# Autodesk Inventor assembly: temp
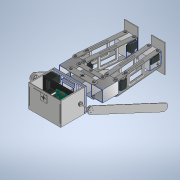
[picture p0: Inventor's stored thumbnail of the model, 180x180]
Saved by Autodesk Inventor 2022 (Build 260153000, 153)
## iProperties
Created: 2022-10-09
Part Number: temp
Document SubType Name: Assembly
Designer: haya
Author: haya
## Documents named in this file (48)
- C:\Users\haya\Documents\GitHub\reduce_joint\reduce_joint.iam
- C:\Users\haya\Documents\GitHub\reduce_joint\foot_link.ipt
- C:\Users\haya\Documents\GitHub\reduce_joint\B3M10xx.ipt
- B3M11xx.ipt
- C:\Users\haya\Documents\GitHub\reduce_joint\ankle.ipt
- C:\Users\haya\Documents\GitHub\reduce_joint\CC-2230-25B.ipt
- C:\Users\haya\Documents\GitHub\reduce_joint\CC-2230-10B.ipt
- C:\Users\haya\Documents\GitHub\reduce_joint\foot.ipt
- C:\Users\haya\Documents\GitHub\reduce_joint\hip.ipt
- C:\Users\haya\Documents\GitHub\reduce_joint\hip_servo_jig.ipt
- C:\Users\haya\Documents\GitHub\reduce_joint\hip_link.ipt
- C:\Users\haya\Documents\GitHub\reduce_joint\crotch.ipt
- C:\Users\haya\Documents\GitHub\reduce_joint\joint.iam
- C:\Users\haya\Documents\GitHub\reduce_joint\waist1..ipt
- C:\Users\haya\Documents\GitHub\reduce_joint\waist2.ipt
- C:\Users\haya\Documents\GitHub\reduce_joint\GEFHBS0_5-50-3-10-W0_b.ipt
- C:\Users\haya\Documents\GitHub\reduce_joint\GEABS0_5-80-2-B-5_b.ipt
- C:\Users\haya\Documents\GitHub\reduce_joint\80F-0505.ipt
- C:\Users\haya\Documents\GitHub\reduce_joint\arm_shaft.ipt
- C:\Users\haya\Documents\GitHub\reduce_joint\body_left.ipt
- C:\Users\haya\Documents\GitHub\reduce_joint\body_right.ipt
- C:\Users\haya\Documents\GitHub\reduce_joint\SSCSJ5-6b.ipt
- C:\Users\haya\Documents\GitHub\reduce_joint\既製品\バッテリー(G7 HI-VOLTAGE 2400MAH 3S 75CMAX LIPO).ipt
- C:\Users\haya\Documents\GitHub\reduce_joint\body_top.ipt
- C:\Users\haya\Documents\GitHub\reduce_joint\raspberrypi_b_+_(assembly)\raspberrypi_b_+_(assembly).iam
- C:\Users\haya\Documents\GitHub\reduce_joint\circuit_base.ipt
- C:\Users\haya\Documents\GitHub\reduce_joint\SCMW5b.ipt
- C:\Users\haya\Documents\GitHub\reduce_joint\arm_link.ipt
- C:\Users\haya\Documents\GitHub\reduce_joint\head.ipt
- C:\Users\haya\Documents\GitHub\reduce_joint\center_servo_jig.ipt
- C:\Users\haya\Documents\GitHub\reduce_joint\lever.ipt
- C:\Users\haya\Documents\GitHub\reduce_joint\foot_link_lever.ipt
- C:\Users\haya\Documents\GitHub\reduce_joint\joint_hip.iam
- C:\Users\haya\Documents\GitHub\reduce_joint\hip_link_motor.ipt
- C:\Users\haya\Documents\GitHub\reduce_joint\foot_connect.ipt
- C:\Users\haya\Documents\GitHub\reduce_joint\foot_link_lever_MIR.ipt
- C:\Users\haya\Documents\GitHub\reduce_joint\B3M10xx_MIR.ipt
- C:\Users\haya\Documents\GitHub\reduce_joint\ankle_MIR.ipt
- C:\Users\haya\Documents\GitHub\reduce_joint\CC-2230-25B_MIR.ipt
- C:\Users\haya\Documents\GitHub\reduce_joint\CC-2230-10B_MIR.ipt
- C:\Users\haya\Documents\GitHub\reduce_joint\foot_MIR.ipt
- C:\Users\haya\Documents\GitHub\reduce_joint\hip_MIR2.ipt
- C:\Users\haya\Documents\GitHub\reduce_joint\foot_link_MIR.ipt
- C:\Users\haya\Documents\GitHub\reduce_joint\hip_servo_jig_MIR.ipt
- C:\Users\haya\Documents\GitHub\reduce_joint\joint_MIR.iam
- C:\Users\haya\Documents\GitHub\reduce_joint\lever_MIR.ipt
- C:\Users\haya\Documents\GitHub\reduce_joint\joint_hip_MIR.iam
- C:\Users\haya\Documents\GitHub\reduce_joint\foot_connect_MIR.ipt
## Components (87 placed, 46 different names)
1. foot_link_lever:1 — 角度:6, 挿入:110, 挿入:111, 正接:1, フラッシュ:16, メイト:26, 角度:11
2. B3M11xx:1 — 角度:1, 挿入:4, 挿入:7
3. ankle:1 — 角度:1, 挿入:4, 挿入:5, 挿入:81, 挿入:82, 角度:2, 挿入:113, 挿入:114
4. CC-2230-25B:1 — 挿入:5, 挿入:6
5. CC-2230-10B:1 — 挿入:6
6. foot:1 — 挿入:7, 角度:2
7. hip:1 — メイト:1, フラッシュ:1, メイト:2, 挿入:77, 挿入:78, 挿入:85, 挿入:86, 角度:6, 挿入:116, 挿入:118, 挿入:121, 挿入:122, 角度:11
8. foot_link:2 — 挿入:84, 挿入:88, メイト:28
9. B3M11xx:2 — フラッシュ:2, メイト:3, フラッシュ:3, 挿入:109
10. hip_servo_jig:1 — メイト:1, フラッシュ:1, メイト:2, フラッシュ:2, メイト:3, フラッシュ:3
11. hip_link:1 — 挿入:72, 挿入:76, 挿入:80, 角度:10
12. hip_link_motor:1 — 挿入:71, 挿入:79, メイト:8
13. crotch:1 — 挿入:74, フラッシュ:4, メイト:4, メイト:5, メイト:7, メイト:8, 角度:3, メイト:9, フラッシュ:5, メイト:10, メイト:11, フラッシュ:6, メイト:12, 挿入:123, 挿入:124, 角度:10
14. joint:1 [sub-assembly] — 挿入:71, 挿入:153
15. joint:2 [sub-assembly] — 挿入:72, 挿入:154
16. joint:3 [sub-assembly] — 挿入:74, 挿入:76
17. joint:4 [sub-assembly] — 挿入:77, 挿入:79
18. joint:6 [sub-assembly] — 挿入:78, 挿入:80
19. joint:7 [sub-assembly] — 挿入:82, 挿入:84
20. joint:8 [sub-assembly] — 挿入:81, 挿入:110
21. joint:9 [sub-assembly] — 挿入:86, 挿入:88
22. joint:10 [sub-assembly] — 挿入:85, 挿入:111
23. B3M11xx:3 — メイト:6, メイト:7, 角度:3
24. center_servo_jig:1 — フラッシュ:4, メイト:4, メイト:5, メイト:6
25. waist1.:1 — メイト:11, フラッシュ:6, メイト:12, メイト:17, フラッシュ:11
26. waist2:1 — メイト:9, フラッシュ:5, メイト:10, メイト:13, フラッシュ:7, フラッシュ:8, メイト:15, メイト:16, フラッシュ:9, フラッシュ:10, フラッシュ:14, メイト:21, 角度:13
27. body_left:1 — メイト:13, フラッシュ:7, フラッシュ:8, 挿入:92, 挿入:93, 挿入:94, 挿入:96, メイト:19, フラッシュ:12, フラッシュ:13, メイト:20
28. B3M11xx:4 — メイト:15, 挿入:94, 挿入:95
29. GEFHBS0_5-50-3-10-W0_b:1 — 挿入:95
30. GEABS0_5-80-2-B-5_b:1 — 挿入:92
31. 80F-0505:1 — 挿入:93
32. arm_shaft:1 — 挿入:96, 挿入:100, 挿入:105
33. body_right:1 — メイト:16, フラッシュ:9, フラッシュ:10, 挿入:97, メイト:18, メイト:23
34. 80F-0505:2 — 挿入:97, 挿入:98
35. SSCSJ5-6b:1 — 挿入:98
36. バッテリー(G7 HI-VOLTAGE 2400MAH 3S 75CMAX LIPO):1 — メイト:17, フラッシュ:11, メイト:18
37. body_top:1 — メイト:19, フラッシュ:12, フラッシュ:13, 挿入:99, 角度:4
38. raspberrypi_b_+_(assembly):1 [sub-assembly] — メイト:22, フラッシュ:15, メイト:23
39. circuit_base:1 — フラッシュ:14, メイト:20, メイト:21, メイト:22, フラッシュ:15
40. B3M11xx:5 — 挿入:99, 角度:4, 挿入:103, 挿入:104
41. SCMW5b:1 — 挿入:100, メイト:24, 挿入:101, 挿入:102
42. arm_link:1 — メイト:24, 挿入:101, 挿入:102, 角度:5
43. head:1 — 挿入:103, 挿入:104
44. SCMW5b:2 — 挿入:105, 挿入:106, 挿入:107
45. arm_link:2 — 挿入:106, 挿入:107, 角度:5, 角度:13
46. lever:1 — 挿入:109, 挿入:112
47. joint_hip:1 [sub-assembly] — 挿入:112, 正接:1
48. joint:11 [sub-assembly] — 挿入:113, 挿入:115
49. joint:12 [sub-assembly] — 挿入:114, 挿入:119
50. foot_link:3 — 挿入:115, 挿入:117, メイト:25
51. joint:13 [sub-assembly] — 挿入:116, 挿入:117
52. foot_connect:1 — メイト:25, フラッシュ:16, メイト:26
53. foot_link:4 — 挿入:119, 挿入:120, フラッシュ:17, メイト:27
54. joint:14 [sub-assembly] — 挿入:118, 挿入:120
55. foot_connect:2 — フラッシュ:17, メイト:27, メイト:28
56. joint:15 [sub-assembly] — 挿入:122, 挿入:129
57. joint:16 [sub-assembly] — 挿入:124, 挿入:130
58. joint:17 [sub-assembly] — 挿入:121, 挿入:127
59. joint:18 [sub-assembly] — 挿入:123, 挿入:128
60. joint:19 [sub-assembly] — 挿入:155
61. joint:20 [sub-assembly] — 挿入:156
62. hip_link:2 — 挿入:127, 挿入:128
63. hip_link:3 — 挿入:129, 挿入:130
64. foot_link_lever_MIR:1 — 角度:9, 挿入:137, 挿入:141, 正接:2, メイト:32, フラッシュ:21, 角度:12
65. B3M10xx_MIR:1 — 挿入:131, 角度:7, 挿入:134
66. ankle_MIR:1 — 挿入:131, 角度:7, 挿入:132, 角度:8, 挿入:136, 挿入:138, 挿入:145, 挿入:146
67. CC-2230-25B_MIR:1 — 挿入:132, 挿入:133
68. CC-2230-10B_MIR:1 — 挿入:133
69. foot_MIR:1 — 角度:8, 挿入:134
70. hip_MIR2:1 — 角度:9, メイト:30, フラッシュ:20, メイト:31, 挿入:140, 挿入:142, 挿入:149, 挿入:152, 挿入:153, 挿入:154, 挿入:155, 挿入:156, 角度:12
71. foot_link_MIR:1 — 挿入:135, 挿入:139, メイト:34
72. B3M10xx_MIR:2 — フラッシュ:18, メイト:29, フラッシュ:19, 挿入:143
73. hip_servo_jig_MIR:1 — フラッシュ:18, メイト:29, フラッシュ:19, メイト:30, フラッシュ:20, メイト:31
74. joint_MIR:1 [sub-assembly] — 挿入:135, 挿入:136
75. joint_MIR:2 [sub-assembly] — 挿入:137, 挿入:138
76. joint_MIR:3 [sub-assembly] — 挿入:139, 挿入:140
77. joint_MIR:4 [sub-assembly] — 挿入:141, 挿入:142
78. lever_MIR:1 — 挿入:143, 挿入:144
79. joint_hip_MIR:1 [sub-assembly] — 正接:2, 挿入:144
80. joint_MIR:5 [sub-assembly] — 挿入:145, 挿入:147
81. joint_MIR:6 [sub-assembly] — 挿入:146, 挿入:150
82. foot_link_MIR:2 — 挿入:147, 挿入:148, メイト:33
83. joint_MIR:7 [sub-assembly] — 挿入:148, 挿入:149
84. foot_connect_MIR:1 — メイト:32, フラッシュ:21, メイト:33
85. foot_link_MIR:3 — 挿入:150, 挿入:151, メイト:35, フラッシュ:22
86. joint_MIR:8 [sub-assembly] — 挿入:151, 挿入:152
87. foot_connect_MIR:2 — メイト:34, メイト:35, フラッシュ:22
## Relationships (151: Insert 80, Mate 34, Flush 22, Angle 13, Tangent 2)
- 角度:1 [Angle] (0 deg): B3M11xx:1 ↔ ankle:1
- 挿入:4 [Insert]: B3M11xx:1 ↔ ankle:1
- 挿入:5 [Insert]: ankle:1 ↔ CC-2230-25B:1
- 挿入:6 [Insert]: CC-2230-25B:1 ↔ CC-2230-10B:1
- 挿入:7 [Insert]: B3M11xx:1 ↔ foot:1
- メイト:1 [Mate]: hip:1 ↔ hip_servo_jig:1
- フラッシュ:1 [Flush] (20 mm): hip:1 ↔ hip_servo_jig:1
- メイト:2 [Mate] (0.5 mm): hip:1 ↔ hip_servo_jig:1
- フラッシュ:2 [Flush]: B3M11xx:2 ↔ hip_servo_jig:1
- メイト:3 [Mate]: B3M11xx:2 ↔ hip_servo_jig:1
- フラッシュ:3 [Flush] (-8.5 mm): B3M11xx:2 ↔ hip_servo_jig:1
- 挿入:71 [Insert]: hip_link_motor:1 ↔ joint:1
- 挿入:72 [Insert]: hip_link:1 ↔ joint:2
- 挿入:74 [Insert]: crotch:1 ↔ joint:3
- 挿入:76 [Insert]: hip_link:1 ↔ joint:3
- 挿入:77 [Insert]: hip:1 ↔ joint:4
- 挿入:78 [Insert]: hip:1 ↔ joint:6
- 挿入:79 [Insert]: hip_link_motor:1 ↔ joint:4
- 挿入:80 [Insert]: hip_link:1 ↔ joint:6
- 挿入:81 [Insert]: ankle:1 ↔ joint:8
- 挿入:82 [Insert]: ankle:1 ↔ joint:7
- 挿入:84 [Insert]: foot_link:2 ↔ joint:7
- 挿入:85 [Insert]: hip:1 ↔ joint:10
- 挿入:86 [Insert]: hip:1 ↔ joint:9
- 挿入:88 [Insert]: foot_link:2 ↔ joint:9
- 角度:2 [Angle] (0 deg): ankle:1 ↔ foot:1
- フラッシュ:4 [Flush]: crotch:1 ↔ center_servo_jig:1
- メイト:4 [Mate]: crotch:1 ↔ center_servo_jig:1
- メイト:5 [Mate] (0.5 mm): crotch:1 ↔ center_servo_jig:1
- メイト:6 [Mate]: B3M11xx:3 ↔ center_servo_jig:1
- メイト:7 [Mate]: crotch:1 ↔ B3M11xx:3
- メイト:8 [Mate]: hip_link_motor:1 ↔ crotch:1
- 角度:3 [Angle] (0 deg): crotch:1 ↔ B3M11xx:3
- メイト:9 [Mate]: crotch:1 ↔ waist2:1
- フラッシュ:5 [Flush]: crotch:1 ↔ waist2:1
- メイト:10 [Mate]: crotch:1 ↔ waist2:1
- メイト:11 [Mate]: crotch:1 ↔ waist1.:1
- フラッシュ:6 [Flush]: crotch:1 ↔ waist1.:1
- メイト:12 [Mate]: crotch:1 ↔ waist1.:1
- メイト:13 [Mate]: waist2:1 ↔ body_left:1
- フラッシュ:7 [Flush]: waist2:1 ↔ body_left:1
- フラッシュ:8 [Flush]: waist2:1 ↔ body_left:1
- メイト:15 [Mate]: waist2:1 ↔ B3M11xx:4
- 挿入:92 [Insert] (1 mm): body_left:1 ↔ GEABS0_5-80-2-B-5_b:1
- 挿入:93 [Insert]: body_left:1 ↔ 80F-0505:1
- 挿入:94 [Insert]: body_left:1 ↔ B3M11xx:4
- 挿入:95 [Insert]: B3M11xx:4 ↔ GEFHBS0_5-50-3-10-W0_b:1
- 挿入:96 [Insert] (-50 mm): body_left:1 ↔ arm_shaft:1
- メイト:16 [Mate]: waist2:1 ↔ body_right:1
- フラッシュ:9 [Flush]: waist2:1 ↔ body_right:1
- フラッシュ:10 [Flush]: waist2:1 ↔ body_right:1
- 挿入:97 [Insert]: body_right:1 ↔ 80F-0505:2
- 挿入:98 [Insert]: 80F-0505:2 ↔ SSCSJ5-6b:1
- メイト:17 [Mate]: waist1.:1 ↔ バッテリー(G7 HI-VOLTAGE 2400MAH 3S 75CMAX LIPO):1
- フラッシュ:11 [Flush] (5 mm): waist1.:1 ↔ バッテリー(G7 HI-VOLTAGE 2400MAH 3S 75CMAX LIPO):1
- メイト:18 [Mate] (10 mm): body_right:1 ↔ バッテリー(G7 HI-VOLTAGE 2400MAH 3S 75CMAX LIPO):1
- メイト:19 [Mate]: body_left:1 ↔ body_top:1
- フラッシュ:12 [Flush]: body_left:1 ↔ body_top:1
- フラッシュ:13 [Flush]: body_left:1 ↔ body_top:1
- フラッシュ:14 [Flush]: waist2:1 ↔ circuit_base:1
- メイト:20 [Mate]: body_left:1 ↔ circuit_base:1
- メイト:21 [Mate] (40 mm): waist2:1 ↔ circuit_base:1
- メイト:22 [Mate] (5 mm): raspberrypi_b_+_(assembly):1 ↔ circuit_base:1
- フラッシュ:15 [Flush]: raspberrypi_b_+_(assembly):1 ↔ circuit_base:1
- 挿入:99 [Insert]: body_top:1 ↔ B3M11xx:5
- 角度:4 [Angle] (0 deg): body_top:1 ↔ B3M11xx:5
- メイト:23 [Mate] (10 mm): body_right:1 ↔ raspberrypi_b_+_(assembly):1
- 挿入:100 [Insert]: arm_shaft:1 ↔ SCMW5b:1
- メイト:24 [Mate]: SCMW5b:1 ↔ arm_link:1
- 挿入:101 [Insert]: SCMW5b:1 ↔ arm_link:1
- 挿入:102 [Insert]: SCMW5b:1 ↔ arm_link:1
- 挿入:103 [Insert]: B3M11xx:5 ↔ head:1
- 挿入:104 [Insert]: B3M11xx:5 ↔ head:1
- 挿入:105 [Insert]: arm_shaft:1 ↔ SCMW5b:2
- 挿入:106 [Insert]: SCMW5b:2 ↔ arm_link:2
- 挿入:107 [Insert]: SCMW5b:2 ↔ arm_link:2
- 角度:5 [Angle] (0 deg): arm_link:1 ↔ arm_link:2
- 角度:6 [Angle] (0 deg): foot_link_lever:1 ↔ hip:1
- 挿入:109 [Insert]: B3M11xx:2 ↔ lever:1
- 挿入:110 [Insert]: foot_link_lever:1 ↔ joint:8
- 挿入:111 [Insert]: foot_link_lever:1 ↔ joint:10
- 挿入:112 [Insert]: lever:1 ↔ joint_hip:1
- 正接:1 [Tangent]: foot_link_lever:1 ↔ joint_hip:1
- 挿入:113 [Insert]: ankle:1 ↔ joint:11
- 挿入:114 [Insert]: ankle:1 ↔ joint:12
- 挿入:115 [Insert]: joint:11 ↔ foot_link:3
- 挿入:116 [Insert]: hip:1 ↔ joint:13
- 挿入:117 [Insert]: foot_link:3 ↔ joint:13
- メイト:25 [Mate]: foot_link:3 ↔ foot_connect:1
- フラッシュ:16 [Flush] (-6.5 mm): foot_link_lever:1 ↔ foot_connect:1
- メイト:26 [Mate] (64 mm): foot_link_lever:1 ↔ foot_connect:1
- 挿入:118 [Insert]: hip:1 ↔ joint:14
- 挿入:119 [Insert]: joint:12 ↔ foot_link:4
- 挿入:120 [Insert]: foot_link:4 ↔ joint:14
- フラッシュ:17 [Flush] (-6.5 mm): foot_link:4 ↔ foot_connect:2
- メイト:27 [Mate]: foot_link:4 ↔ foot_connect:2
- メイト:28 [Mate] (64 mm): foot_link:2 ↔ foot_connect:2
- 挿入:121 [Insert]: hip:1 ↔ joint:17
- 挿入:122 [Insert]: hip:1 ↔ joint:15
- 挿入:123 [Insert]: crotch:1 ↔ joint:18
- 挿入:124 [Insert]: crotch:1 ↔ joint:16
- 挿入:127 [Insert]: joint:17 ↔ hip_link:2
- 挿入:128 [Insert]: joint:18 ↔ hip_link:2
- 挿入:129 [Insert]: joint:15 ↔ hip_link:3
- 挿入:130 [Insert]: joint:16 ↔ hip_link:3
- 挿入:131 [Insert]: B3M10xx_MIR:1 ↔ ankle_MIR:1
- 角度:7 [Angle] (0 deg): B3M10xx_MIR:1 ↔ ankle_MIR:1
- 挿入:132 [Insert]: ankle_MIR:1 ↔ CC-2230-25B_MIR:1
- 挿入:133 [Insert]: CC-2230-25B_MIR:1 ↔ CC-2230-10B_MIR:1
- 角度:8 [Angle] (0 deg): ankle_MIR:1 ↔ foot_MIR:1
- 挿入:134 [Insert]: B3M10xx_MIR:1 ↔ foot_MIR:1
- 角度:9 [Angle] (0 deg): foot_link_lever_MIR:1 ↔ hip_MIR2:1
- フラッシュ:18 [Flush] (-8.5 mm): B3M10xx_MIR:2 ↔ hip_servo_jig_MIR:1
- メイト:29 [Mate]: B3M10xx_MIR:2 ↔ hip_servo_jig_MIR:1
- フラッシュ:19 [Flush]: B3M10xx_MIR:2 ↔ hip_servo_jig_MIR:1
- メイト:30 [Mate] (0.5 mm): hip_MIR2:1 ↔ hip_servo_jig_MIR:1
- フラッシュ:20 [Flush] (20 mm): hip_MIR2:1 ↔ hip_servo_jig_MIR:1
- メイト:31 [Mate]: hip_MIR2:1 ↔ hip_servo_jig_MIR:1
- 挿入:135 [Insert]: foot_link_MIR:1 ↔ joint_MIR:1
- 挿入:136 [Insert]: ankle_MIR:1 ↔ joint_MIR:1
- 挿入:137 [Insert]: foot_link_lever_MIR:1 ↔ joint_MIR:2
- 挿入:138 [Insert]: ankle_MIR:1 ↔ joint_MIR:2
- 挿入:139 [Insert]: foot_link_MIR:1 ↔ joint_MIR:3
- 挿入:140 [Insert]: hip_MIR2:1 ↔ joint_MIR:3
- 挿入:141 [Insert]: foot_link_lever_MIR:1 ↔ joint_MIR:4
- 挿入:142 [Insert]: hip_MIR2:1 ↔ joint_MIR:4
- 挿入:143 [Insert]: B3M10xx_MIR:2 ↔ lever_MIR:1
- 正接:2 [Tangent]: foot_link_lever_MIR:1 ↔ joint_hip_MIR:1
- 挿入:144 [Insert]: lever_MIR:1 ↔ joint_hip_MIR:1
- 挿入:145 [Insert]: ankle_MIR:1 ↔ joint_MIR:5
- 挿入:146 [Insert]: ankle_MIR:1 ↔ joint_MIR:6
- 挿入:147 [Insert]: joint_MIR:5 ↔ foot_link_MIR:2
- 挿入:148 [Insert]: foot_link_MIR:2 ↔ joint_MIR:7
- 挿入:149 [Insert]: hip_MIR2:1 ↔ joint_MIR:7
- メイト:32 [Mate] (64 mm): foot_link_lever_MIR:1 ↔ foot_connect_MIR:1
- フラッシュ:21 [Flush] (-6.5 mm): foot_link_lever_MIR:1 ↔ foot_connect_MIR:1
- メイト:33 [Mate]: foot_link_MIR:2 ↔ foot_connect_MIR:1
- 挿入:150 [Insert]: joint_MIR:6 ↔ foot_link_MIR:3
- 挿入:151 [Insert]: foot_link_MIR:3 ↔ joint_MIR:8
- 挿入:152 [Insert]: hip_MIR2:1 ↔ joint_MIR:8
- メイト:34 [Mate] (64 mm): foot_link_MIR:1 ↔ foot_connect_MIR:2
- メイト:35 [Mate]: foot_link_MIR:3 ↔ foot_connect_MIR:2
- フラッシュ:22 [Flush] (-6.5 mm): foot_link_MIR:3 ↔ foot_connect_MIR:2
- 挿入:153 [Insert]: joint:1 ↔ hip_MIR2:1
- 挿入:154 [Insert]: joint:2 ↔ hip_MIR2:1
- 挿入:155 [Insert]: joint:19 ↔ hip_MIR2:1
- 挿入:156 [Insert]: joint:20 ↔ hip_MIR2:1
- 角度:10 [Angle] (0 deg): hip_link:1 ↔ crotch:1
- 角度:11 [Angle] (5 deg): foot_link_lever:1 ↔ hip:1
- 角度:12 [Angle] (-5 deg): foot_link_lever_MIR:1 ↔ hip_MIR2:1
- 角度:13 [Angle] (25 deg): waist2:1 ↔ arm_link:2
